# Autodesk Inventor assembly: Ensamblaje carcasa control
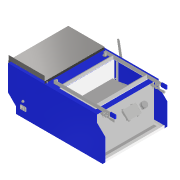
[picture p0: Inventor's stored thumbnail of the model, 180x180]
Saved by Autodesk Inventor 2021 (Build 250183000, 183)
## iProperties
Created: 2021-04-15
Part Number: Ensamblaje carcasa control
Document SubType Name: Assembly
Designer: Admin
Author: Admin
## Documents named in this file (19)
- C:\Users\carlo\Desktop\Pai\Proyecto_PAI_2021\01 CAD\Ensamblaje carcasa control.iam
- C:\Users\carlo\Desktop\Pai\Proyecto_PAI_2021\01 CAD\Carcasa_azul.ipt
- C:\Users\carlo\Desktop\Pai\Proyecto_PAI_2021\01 CAD\Carcaza_blanca_frontal.ipt
- C:\Users\carlo\Desktop\Pai\Proyecto_PAI_2021\01 CAD\Tapa_blanca_inferior.ipt
- C:\Users\carlo\Desktop\Pai\Proyecto_PAI_2021\01 CAD\Vacuometro.ipt
- C:\Users\carlo\Desktop\Pai\Proyecto_PAI_2021\01 CAD\HMI_NV3W_MR20L_V1.iam
- C:\Users\carlo\Desktop\Pai\Proyecto_PAI_2021\01 CAD\Receptaculo e interruptor.ipt
- C:\Users\carlo\Desktop\Pai\Proyecto_PAI_2021\01 CAD\Portafusible para fusible de 13A.ipt
- C:\Users\carlo\Desktop\Pai\Proyecto_PAI_2021\01 CAD\Tapa_interior_1.ipt
- C:\Users\carlo\Desktop\Pai\Proyecto_PAI_2021\01 CAD\Tapa_interior_2.ipt
- C:\Users\carlo\Desktop\Pai\Proyecto_PAI_2021\01 CAD\Tapa_blanca_trasera.ipt
- C:\Users\carlo\Desktop\Pai\Proyecto_PAI_2021\01 CAD\Ensamble eléctrico.iam
- C:\Users\carlo\Desktop\Pai\Proyecto_PAI_2021\01 CAD\Bomba de Vacio.ipt
- C:\Users\carlo\Desktop\Pai\Proyecto_PAI_2021\01 CAD\Marco molde.ipt
- C:\Users\carlo\Desktop\Pai\Proyecto_PAI_2021\01 CAD\CSN 02 1721 - 17,5.ipt
- C:\Users\carlo\Desktop\Pai\Proyecto_PAI_2021\01 CAD\Ensamblaje_soportme molde_barras.iam
- C:\Users\carlo\Desktop\Pai\Proyecto_PAI_2021\01 CAD\Mecanismo Modelado.iam
- C:\Users\carlo\Desktop\Pai\Proyecto_PAI_2021\01 CAD\Bandeja_proteccion_carcasa_control.ipt
- C:\Users\carlo\Desktop\Pai\Proyecto_PAI_2021\01 CAD\MecanismoBoqueoCarro\ProtectorBloqueo.ipt
## Components (19 placed, 18 different names)
1. Carcasa_azul:1 — Coincidencia:1, Nivelación:1, Coincidencia:2, Coincidencia:3, Nivelación:2, Coincidencia:5, Coincidencia:6, Coincidencia:7, Coincidencia:8, Coincidencia:9, Coincidencia:15, Coincidencia:16, Coincidencia:18, Coincidencia:20, Coincidencia:27, Nivelación:6, Nivelación:7, Coincidencia:28, Coincidencia:29, Coincidencia:30, Coincidencia:31, Coincidencia:32, Coincidencia:34, Nivelación:8, Nivelación:9, Coincidencia:35, Mate:36, Mate:37
2. Carcaza_blanca_frontal:1 — Coincidencia:1, Nivelación:1, Coincidencia:2, Coincidencia:4, Coincidencia:10, Coincidencia:11, Coincidencia:12, Coincidencia:13, Coincidencia:14, Coincidencia:19
3. Tapa_blanca_inferior:1 — Coincidencia:3, Coincidencia:4, Nivelación:2, Nivelación:4, Coincidencia:21, Mate:25, Flush:5, Mate:26
4. Vacuometro:1 — Coincidencia:10, Coincidencia:11
5. HMI_NV3W_MR20L_V1:1 [sub-assembly] — Coincidencia:12, Coincidencia:13, Coincidencia:14
6. Receptaculo e interruptor:1 — Coincidencia:7, Coincidencia:8, Coincidencia:9
7. Portafusible para fusible de 13A:1 — Coincidencia:5, Coincidencia:6
8. Tapa_interior_1:1 — Coincidencia:15, Coincidencia:16, Nivelación:3, Mate:22, Mate:23, Mate:24
9. Tapa_interior_2:1 — Coincidencia:18, Coincidencia:19, Nivelación:3
10. Tapa_blanca_trasera:1 — Coincidencia:20, Nivelación:4, Coincidencia:21
11. Ensamble eléctrico:1 [sub-assembly] — Mate:22, Mate:23, Mate:24
12. Bomba de Vacio:1 — Mate:25, Flush:5, Mate:26
13. Marco molde:1 — Coincidencia:27, Nivelación:6, Nivelación:7
14. CSN 02 1721 17,5:1 — Coincidencia:28, Coincidencia:30, Cilíndrica:1
15. CSN 02 1721 17,5:2 — Coincidencia:29, Coincidencia:31
16. Ensamblaje_soportme molde_barras:1 [sub-assembly] — Cilíndrica:1
17. Mecanismo Modelado:1 [sub-assembly] — Coincidencia:32, Coincidencia:34
18. Bandeja_proteccion_carcasa_control:1 — Nivelación:8, Nivelación:9, Coincidencia:35
19. ProtectorBloqueo:1 — Mate:36, Mate:37
## Relationships (45: Mate 35, Flush 9, CylindricalJoint 1)
- Coincidencia:1 [Mate]: Carcasa_azul:1 ↔ Carcaza_blanca_frontal:1
- Nivelación:1 [Flush]: Carcasa_azul:1 ↔ Carcaza_blanca_frontal:1
- Coincidencia:2 [Mate]: Carcasa_azul:1 ↔ Carcaza_blanca_frontal:1
- Coincidencia:3 [Mate]: Carcasa_azul:1 ↔ Tapa_blanca_inferior:1
- Coincidencia:4 [Mate]: Carcaza_blanca_frontal:1 ↔ Tapa_blanca_inferior:1
- Nivelación:2 [Flush]: Carcasa_azul:1 ↔ Tapa_blanca_inferior:1
- Coincidencia:5 [Mate]: Carcasa_azul:1 ↔ Portafusible para fusible de 13A:1
- Coincidencia:6 [Mate]: Carcasa_azul:1 ↔ Portafusible para fusible de 13A:1
- Coincidencia:7 [Mate]: Carcasa_azul:1 ↔ Receptaculo e interruptor:1
- Coincidencia:8 [Mate]: Carcasa_azul:1 ↔ Receptaculo e interruptor:1
- Coincidencia:9 [Mate]: Carcasa_azul:1 ↔ Receptaculo e interruptor:1
- Coincidencia:10 [Mate]: Carcaza_blanca_frontal:1 ↔ Vacuometro:1
- Coincidencia:11 [Mate]: Carcaza_blanca_frontal:1 ↔ Vacuometro:1
- Coincidencia:12 [Mate]: Carcaza_blanca_frontal:1 ↔ HMI_NV3W_MR20L_V1:1
- Coincidencia:13 [Mate]: Carcaza_blanca_frontal:1 ↔ HMI_NV3W_MR20L_V1:1
- Coincidencia:14 [Mate]: Carcaza_blanca_frontal:1 ↔ HMI_NV3W_MR20L_V1:1
- Coincidencia:15 [Mate]: Carcasa_azul:1 ↔ Tapa_interior_1:1
- Coincidencia:16 [Mate] (20 mm): Carcasa_azul:1 ↔ Tapa_interior_1:1
- Coincidencia:18 [Mate]: Carcasa_azul:1 ↔ Tapa_interior_2:1
- Coincidencia:19 [Mate]: Carcaza_blanca_frontal:1 ↔ Tapa_interior_2:1
- Nivelación:3 [Flush]: Tapa_interior_1:1 ↔ Tapa_interior_2:1
- Coincidencia:20 [Mate]: Carcasa_azul:1 ↔ Tapa_blanca_trasera:1
- Nivelación:4 [Flush]: Tapa_blanca_inferior:1 ↔ Tapa_blanca_trasera:1
- Coincidencia:21 [Mate]: Tapa_blanca_inferior:1 ↔ Tapa_blanca_trasera:1
- Mate:22: Tapa_interior_1:1 ↔ Ensamble eléctrico:1
- Mate:23: Tapa_interior_1:1 ↔ Ensamble eléctrico:1
- Mate:24: Tapa_interior_1:1 ↔ Ensamble eléctrico:1
- Mate:25: Tapa_blanca_inferior:1 ↔ Bomba de Vacio:1
- Flush:5 (70 mm): Tapa_blanca_inferior:1 ↔ Bomba de Vacio:1
- Mate:26 (130 mm): Tapa_blanca_inferior:1 ↔ Bomba de Vacio:1
- Coincidencia:27 [Mate]: Carcasa_azul:1 ↔ Marco molde:1
- Nivelación:6 [Flush]: Carcasa_azul:1 ↔ Marco molde:1
- Nivelación:7 [Flush]: Carcasa_azul:1 ↔ Marco molde:1
- Coincidencia:28 [Mate]: Carcasa_azul:1 ↔ CSN 02 1721 17,5:1
- Coincidencia:29 [Mate]: Carcasa_azul:1 ↔ CSN 02 1721 17,5:2
- Coincidencia:30 [Mate]: Carcasa_azul:1 ↔ CSN 02 1721 17,5:1
- Coincidencia:31 [Mate]: Carcasa_azul:1 ↔ CSN 02 1721 17,5:2
- Cilíndrica:1 [CylindricalJoint]: CSN 02 1721 17,5:1 ↔ Ensamblaje_soportme molde_barras:1
- Coincidencia:32 [Mate]: Carcasa_azul:1 ↔ Mecanismo Modelado:1
- Coincidencia:34 [Mate]: Carcasa_azul:1 ↔ Mecanismo Modelado:1
- Nivelación:8 [Flush] (5 mm): Carcasa_azul:1 ↔ Bandeja_proteccion_carcasa_control:1
- Nivelación:9 [Flush]: Carcasa_azul:1 ↔ Bandeja_proteccion_carcasa_control:1
- Coincidencia:35 [Mate]: Carcasa_azul:1 ↔ Bandeja_proteccion_carcasa_control:1
- Mate:36: Carcasa_azul:1 ↔ ProtectorBloqueo:1
- Mate:37: Carcasa_azul:1 ↔ ProtectorBloqueo:1
